# Autodesk Inventor assembly: ASY PNS780-Filter legs D1200
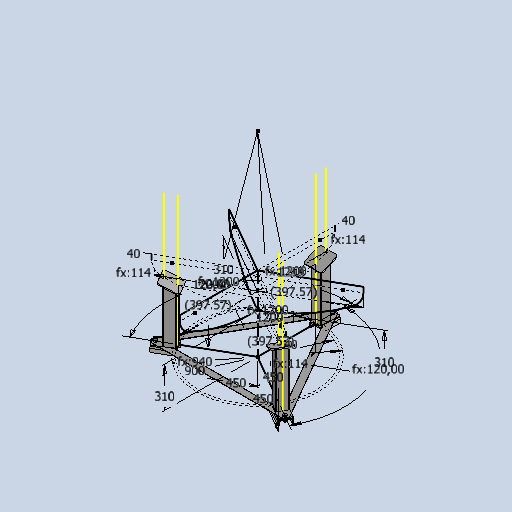
[picture p0: Inventor's stored thumbnail of the model, 512x512]
Saved by Autodesk Inventor 2025.1 (Build 291241020, 241B)
## iProperties
Created: 2025-02-20
Part Number: ASY PNS780-Filter legs D1200
Document SubType Name: Assembly
Designer: user
Author: user
## Documents named in this file (9)
- C:\Users\user\YandexDisk-badmisterfox\home pc\Inventor\PNS-Panaevsk\Filter D1200\ASY PNS780-Filter legs D1200.iam
- C:\Users\user\YandexDisk-badmisterfox\home pc\Inventor\PNS-Panaevsk\Filter D1200\PNS-781 Leg tube.ipt
- C:\Users\user\YandexDisk-badmisterfox\home pc\Inventor\PNS-Panaevsk\Filter D1200\PNS-789 leg sketch.ipt
- C:\Users\user\YandexDisk-badmisterfox\home pc\Inventor\PNS-Panaevsk\Filter D1200\PNS-782 leg plate for filter.ipt
- C:\Users\user\YandexDisk-badmisterfox\home pc\Inventor\PNS-Panaevsk\Filter D1200\PNS-783 leg floor plate.ipt
- C:\Users\user\YandexDisk-badmisterfox\home pc\Inventor\PNS-Panaevsk\Filter D1200\PNS-785 leg floor channel.ipt
- C:\Users\user\YandexDisk-badmisterfox\home pc\Inventor\PNS-Panaevsk\CC\en-US\DIN EN ISO 8673\DIN EN ISO 8673 - M16 x 1.5.ipt
- C:\Users\user\YandexDisk-badmisterfox\home pc\Inventor\PNS-Panaevsk\CC\en-US\ISO 4017(1)\ISO 4017 - M16 x 40 - ISO.ipt
- C:\Users\user\YandexDisk-badmisterfox\home pc\Inventor\PNS-Panaevsk\Filter D1000\PNS-688 leg 1200 pattern.ipt
## Components (20 placed, 8 different names)
1. ISO 4019 - 200x200x5 - 800.ipt:1 — Mate:2, Mate:8, Tangent:2, Rigid:2, Rigid:5
2. ISO 4019 - 200x200x5 - 800.ipt:2 — Mate:4, Mate:7, Tangent:3, Rigid:1, Rigid:4
3. ISO 4019 - 200x200x5 - 800.ipt:3 — Mate:3, Mate:6, Tangent:1, Rigid:3, Rigid:6
4. Part2ntdddasd.ipt:1 — Mate:6, Tangent:1, Mate:7, Mate:8, Tangent:2, Tangent:3
5. temp filter leg plate.ipt:1 — Rigid:1
6. temp filter leg plate.ipt:2 — Rigid:2
7. temp filter leg plate.ipt:3 — Rigid:3
8. temp filter leg plate_CPY.ipt:1 — Rigid:4, Rigid:9, Rotational:3, Rigid:10
9. temp filter leg plate_CPY.ipt:2 — Rigid:5, Rigid:7, Rotational:7
10. temp filter leg plate_CPY.ipt:3 — Rigid:6, Rigid:8, Rotational:5
11. PNS-785 leg floor channel:1 — Rigid:7, Rotational:6
12. PNS-785 leg floor channel:2 — Rigid:9, Rotational:2
13. PNS-785 leg floor channel:3 — Rigid:8, Rotational:4
14. ISO 4017 M16 x 40:1 — Rotational:3
15. DIN EN ISO 8673 M16 x 1.5:1 — Rotational:2
16. DIN EN ISO 8673 M16 x 1.5:2 — Rotational:6
17. ISO 4017 M16 x 40:2 — Rotational:7
18. DIN EN ISO 8673 M16 x 1.5:3 — Rotational:4
19. ISO 4017 M16 x 40:3 — Rotational:5
20. PNS-688 leg 1200 pattern:1 — Rigid:10
## Relationships (25: WeldJoint 10, Mate 6, RevoluteJoint 6, Tangent 3)
- Mate:2: ISO 4019 - 200x200x5 - 800.ipt:1
- Mate:3: ISO 4019 - 200x200x5 - 800.ipt:3
- Mate:4: ISO 4019 - 200x200x5 - 800.ipt:2
- Mate:6: ISO 4019 - 200x200x5 - 800.ipt:3 ↔ Part2ntdddasd.ipt:1
- Tangent:1: ISO 4019 - 200x200x5 - 800.ipt:3 ↔ Part2ntdddasd.ipt:1
- Mate:7: ISO 4019 - 200x200x5 - 800.ipt:2 ↔ Part2ntdddasd.ipt:1
- Mate:8: ISO 4019 - 200x200x5 - 800.ipt:1 ↔ Part2ntdddasd.ipt:1
- Tangent:2: ISO 4019 - 200x200x5 - 800.ipt:1 ↔ Part2ntdddasd.ipt:1
- Tangent:3: ISO 4019 - 200x200x5 - 800.ipt:2 ↔ Part2ntdddasd.ipt:1
- Rigid:1 [WeldJoint]: ISO 4019 - 200x200x5 - 800.ipt:2 ↔ temp filter leg plate.ipt:1
- Rigid:2 [WeldJoint]: ISO 4019 - 200x200x5 - 800.ipt:1 ↔ temp filter leg plate.ipt:2
- Rigid:3 [WeldJoint]: ISO 4019 - 200x200x5 - 800.ipt:3 ↔ temp filter leg plate.ipt:3
- Rigid:4 [WeldJoint]: ISO 4019 - 200x200x5 - 800.ipt:2 ↔ temp filter leg plate_CPY.ipt:1
- Rigid:5 [WeldJoint]: ISO 4019 - 200x200x5 - 800.ipt:1 ↔ temp filter leg plate_CPY.ipt:2
- Rigid:6 [WeldJoint]: ISO 4019 - 200x200x5 - 800.ipt:3 ↔ temp filter leg plate_CPY.ipt:3
- Rigid:7 [WeldJoint]: temp filter leg plate_CPY.ipt:2 ↔ PNS-785 leg floor channel:1
- Rigid:8 [WeldJoint]: temp filter leg plate_CPY.ipt:3 ↔ PNS-785 leg floor channel:3
- Rigid:9 [WeldJoint]: temp filter leg plate_CPY.ipt:1 ↔ PNS-785 leg floor channel:2
- Rotational:2 [RevoluteJoint]: PNS-785 leg floor channel:2 ↔ DIN EN ISO 8673 M16 x 1.5:1
- Rotational:3 [RevoluteJoint]: temp filter leg plate_CPY.ipt:1 ↔ ISO 4017 M16 x 40:1
- Rotational:4 [RevoluteJoint]: PNS-785 leg floor channel:3 ↔ DIN EN ISO 8673 M16 x 1.5:3
- Rotational:5 [RevoluteJoint]: temp filter leg plate_CPY.ipt:3 ↔ ISO 4017 M16 x 40:3
- Rotational:6 [RevoluteJoint]: PNS-785 leg floor channel:1 ↔ DIN EN ISO 8673 M16 x 1.5:2
- Rotational:7 [RevoluteJoint]: temp filter leg plate_CPY.ipt:2 ↔ ISO 4017 M16 x 40:2
- Rigid:10 [WeldJoint]: temp filter leg plate_CPY.ipt:1 ↔ PNS-688 leg 1200 pattern:1
